# Autodesk Inventor assembly: koleso
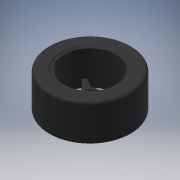
[picture p0: Inventor's stored thumbnail of the model, 180x180]
Saved by Autodesk Inventor 2016 (Build 200138000, 138)
## iProperties
Created: 2016-11-29
Part Number: koleso
Document SubType Name: Assembly
Designer: Juraj
Author: Juraj
## Documents named in this file (3)
- C:\Users\Juraj\Documents\GitHub\Robot6x6\Terrenny robot CAD\koleso\koleso.iam
- C:\Users\Juraj\Documents\GitHub\Robot6x6\Terrenny robot CAD\koleso\koleso.ipt
- C:\Users\Juraj\Documents\GitHub\Robot6x6\Terrenny robot CAD\guma.ipt
## Components (2 placed, 2 different names)
1. koleso:1 — Mate:1, Mate:2
2. guma:1 — Mate:1, Mate:2
## Relationships (2: Mate 2)
- Mate:1: koleso:1 ↔ guma:1
- Mate:2: koleso:1 ↔ guma:1
